# Autodesk Inventor assembly: Assembly_7_button
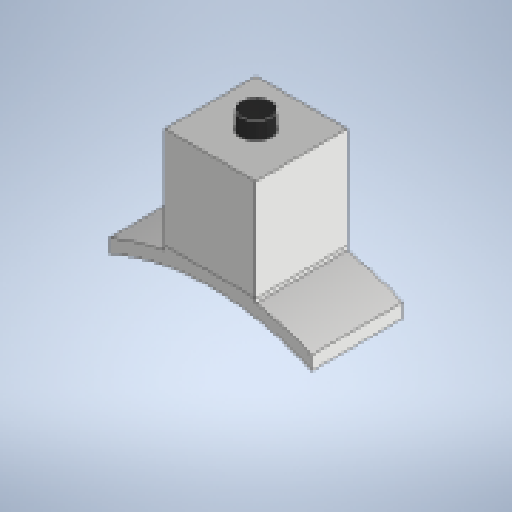
[picture p0: Inventor's stored thumbnail of the model, 512x512]
Saved by Autodesk Inventor 2023 (Build 270158000, 158)
## iProperties
Created: 2023-10-25
Part Number: Assembly_7_button
Document SubType Name: Assembly
Designer: zskus
Author: zskus
## Documents named in this file (4)
- C:\Users\zskus\Desktop\Folders\Personal Projects\Inventor\Project_1_Scooter\Assembly\Assembly_7_button.iam
- C:\Users\zskus\Desktop\Folders\Personal Projects\Inventor\Project_1_Scooter\Parts\BUTTON v1.iam
- C:\Users\zskus\Desktop\Folders\Personal Projects\Inventor\Project_1_Scooter\Parts\button_holder.ipt
- C:\Users\zskus\Desktop\Folders\Personal Projects\Inventor\Project_1_Scooter\Parts\buttonholderscooterpart.ipt
## Components (3 placed, 3 different names)
1. BUTTON v1:1 [sub-assembly] — Mate:1, Mate:2, Angle:1
2. button_holder:1 — Mate:1, Mate:2, Angle:1, Mate:3, Flush:1, Flush:2
3. buttonholderscooterpart:1 — Mate:3, Flush:1, Flush:2
## Relationships (6: Mate 3, Flush 2, Angle 1)
- Mate:1: BUTTON v1:1 ↔ button_holder:1
- Mate:2: BUTTON v1:1 ↔ button_holder:1
- Angle:1 (0 deg): BUTTON v1:1 ↔ button_holder:1
- Mate:3: button_holder:1 ↔ buttonholderscooterpart:1
- Flush:1: button_holder:1 ↔ buttonholderscooterpart:1
- Flush:2: button_holder:1 ↔ buttonholderscooterpart:1
